# Autodesk Inventor assembly: Rocket
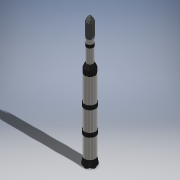
[picture p0: Inventor's stored thumbnail of the model, 180x180]
Saved by Autodesk Inventor 2016 (Build 200138000, 138)
## iProperties
Created: 2016-04-24
Part Number: Rocket
Document SubType Name: Assembly
Designer: etman
Author: etman
## Documents named in this file (12)
- C:\Users\etman\Documents\Rocket.iam
- C:\Users\etman\Documents\Part01.ipt
- C:\Users\etman\Documents\Part02.ipt
- C:\Users\etman\Documents\Part04.ipt
- C:\Users\etman\Documents\Part05.ipt
- C:\Users\etman\Documents\conector.ipt
- C:\Users\etman\Documents\stage2_part1.ipt
- C:\Users\etman\Documents\stage2_part2.ipt
- C:\Users\etman\Documents\stage3_part1.ipt
- C:\Users\etman\Documents\stage3_part2.ipt
- C:\Users\etman\Documents\stage 4.ipt
- C:\Users\etman\Documents\final.ipt
## Components (11 placed, 11 different names)
1. Part01:1 — Rigid:2, Rigid:3, Rigid:4
2. Part02:1 — Rigid:2, Rotational:1, Cylindrical:1
3. Part04:1 — Cylindrical:1
4. Part05:1 — Rotational:1
5. conector:1 — Rigid:3
6. stage2_part1:1 — Rigid:4, Rotational:2
7. stage2_part2:1 — Rotational:2, Rigid:5
8. stage3_part1:1 — Rigid:5, Rigid:6, Rigid:7
9. stage3_part2:1 — Rigid:6
10. stage 4:1 — Rigid:7, Rigid:8
11. final:1 — Rigid:8
## Relationships (10: WeldJoint 7, RevoluteJoint 2, CylindricalJoint 1)
- Rigid:2 [WeldJoint]: Part01:1 ↔ Part02:1
- Rotational:1 [RevoluteJoint]: Part02:1 ↔ Part05:1
- Cylindrical:1: Part02:1 ↔ Part04:1
- Rigid:3 [WeldJoint]: Part01:1 ↔ conector:1
- Rigid:4 [WeldJoint]: Part01:1 ↔ stage2_part1:1
- Rotational:2 [RevoluteJoint]: stage2_part1:1 ↔ stage2_part2:1
- Rigid:5 [WeldJoint]: stage2_part2:1 ↔ stage3_part1:1
- Rigid:6 [WeldJoint]: stage3_part1:1 ↔ stage3_part2:1
- Rigid:7 [WeldJoint]: stage3_part1:1 ↔ stage 4:1
- Rigid:8 [WeldJoint]: stage 4:1 ↔ final:1
